# Autodesk Inventor assembly: 446 Wheel Shaft
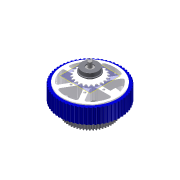
[picture p0: Inventor's stored thumbnail of the model, 180x180]
Saved by Autodesk Inventor 2013 (Build 170138000, 138)
## iProperties
Created: 2012-10-14
Part Number: 446 Wheel Shaft
Document SubType Name: Assembly
Designer: Nemo
Author: Nemo
## Documents named in this file (8)
- H:\Nemo\Documents\Robotics\COTS Parts\Gearboxes\Shafts\446 Wheel Shaft.iam
- H:\Nemo\Documents\Robotics\COTS Parts\Gearboxes\Shafts\446 Cluster Hex Shaft.ipt
- H:\Nemo\Documents\Robotics\COTS Parts\Gearboxes\Bearings\Bearing FR8zz.ipt
- H:\Nemo\Documents\Robotics\COTS Parts\Gearboxes\Spacers\446 wheel spacer.ipt
- H:\Nemo\Documents\Robotics\COTS Parts\Gearboxes\Spacers\446 wheel sprocket spacer.ipt
- H:\Nemo\Documents\Robotics\COTS Parts\Sprockets\25 sprocket 22T 500Hex.ipt
- H:\Nemo\Documents\Robotics\COTS Parts\Wheels\4in Performance Hex Bore nitrile.iam
- H:\Nemo\Documents\Robotics\COTS Parts\Gearboxes\Gears\Gear 20dp 500hex 56T.ipt
## Components (8 placed, 7 different names)
1. 446 Cluster Hex Shaft:1 — Insert:1, Mate:1, Mate:3, Angle:1, Mate:5, Angle:2, Mate:6, Mate:7
2. Bearing FR8zz:1 — Mate:1, Mate:2, Mate:9
3. Bearing FR8zz:2 — Insert:1, Mate:2, Insert:2
4. 446 wheel spacer:1 — Mate:6, Mate:10
5. 446 wheel sprocket spacer:1 — Insert:2, Mate:4
6. 25 Sprocket 22T 500K:1 — Mate:3, Angle:1, Mate:4, Mate:8
7. 4in Performance Hex Bore nitrile:1 [sub-assembly] — Mate:5, Angle:2, Mate:8
8. Gear 56T 20dp 500hex:1 — Mate:7, Mate:9, Mate:10
## Relationships (14: Mate 10, Insert 2, Angle 2)
- Insert:1 (1.0922 mm): 446 Cluster Hex Shaft:1 ↔ Bearing FR8zz:2
- Mate:1: 446 Cluster Hex Shaft:1 ↔ Bearing FR8zz:1
- Mate:2 (-66.04 mm): Bearing FR8zz:1 ↔ Bearing FR8zz:2
- Mate:3: 446 Cluster Hex Shaft:1 ↔ 25 Sprocket 22T 500K:1
- Angle:1 (0 deg): 446 Cluster Hex Shaft:1 ↔ 25 Sprocket 22T 500K:1
- Insert:2: Bearing FR8zz:2 ↔ 446 wheel sprocket spacer:1
- Mate:4: 446 wheel sprocket spacer:1 ↔ 25 Sprocket 22T 500K:1
- Mate:5: 446 Cluster Hex Shaft:1 ↔ 4in Performance Hex Bore nitrile:1
- Angle:2 (0 deg): 446 Cluster Hex Shaft:1 ↔ 4in Performance Hex Bore nitrile:1
- Mate:6: 446 Cluster Hex Shaft:1 ↔ 446 wheel spacer:1
- Mate:7: 446 Cluster Hex Shaft:1 ↔ Gear 56T 20dp 500hex:1
- Mate:8: 25 Sprocket 22T 500K:1 ↔ 4in Performance Hex Bore nitrile:1
- Mate:9: Bearing FR8zz:1 ↔ Gear 56T 20dp 500hex:1
- Mate:10: 446 wheel spacer:1 ↔ Gear 56T 20dp 500hex:1
